# Autodesk Inventor assembly: Блок подъёма первога звена
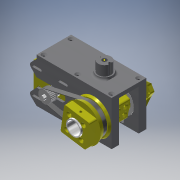
[picture p0: Inventor's stored thumbnail of the model, 180x180]
Saved by Autodesk Inventor 2019.1 (Build 231200000, 200)
## iProperties
Created: 2018-10-15
Part Number: Блок подъёма первога звена
Material: Типовые
Document SubType Name: Assembly
Designer: Олег
Author: Олег
## Documents named in this file (9)
- C:\Users\Олег\OneDrive\Общая\NoSpace 2.0\Манипулятор\Блок подъёма первога звена.iam
- C:\Users\Олег\OneDrive\Общая\NoSpace 2.0\Манипулятор\Основная часть подъемного механизма первого звена.iam
- C:\Users\Олег\OneDrive\Общая\NoSpace 2.0\Мотор-колесо\Мотор\Мотор.iam
- C:\Users\Олег\OneDrive\Общая\NoSpace 2.0\Манипулятор\Ось подъёмного блока первого звена.ipt
- C:\Users\Олег\OneDrive\Общая\NoSpace 2.0\Манипулятор\Переходник от первого звена к оси.ipt
- C:\Users\Олег\OneDrive\Общая\NoSpace 2.0\Манипулятор\Съёмное крепление мотора 37мм.ipt
- C:\Users\Олег\OneDrive\Общая\NoSpace 2.0\Манипулятор\Узел потенциометра.iam
- C:\Users\Олег\OneDrive\Общая\NoSpace 2.0\Манипулятор\Шкив.iam
- C:\Users\Олег\OneDrive\Общая\NoSpace 2.0\Манипулятор\Блок подъёма первога звена\Мастер проектирования\Передача с помощью зубчатых ремней4.iam
## Components (8 placed, 8 different names)
1. Основная часть подъемного механизма первого звена:1 [sub-assembly] — Совмещение:2, Совмещение:6, Заподлицо:1, Совмещение:8, Совмещение:9, Совмещение:10, Совмещение:11, Угол:1
2. Ось подъёмного блока первого звена:1 — Совмещение:6, Заподлицо:1, Совмещение:7, Совмещение:12, Заподлицо:2
3. Переходник от первого звена к оси:1 — Совмещение:7, Совмещение:8, Угол:2
4. Съёмное крепление мотора 37мм:1 — Совмещение:2, Совмещение:3, Совмещение:4, Совмещение:5, Угол:1
5. Узел потенциометра:1 [sub-assembly] — Совмещение:9, Совмещение:10, Совмещение:11
6. Шкив:1 [sub-assembly] — Совмещение:12, Заподлицо:2, Угол:2
7. Мотор:1 [sub-assembly] — Совмещение:3, Совмещение:4, Совмещение:5, Совмещение:13
8. Передача с помощью зубчатых ремней:1 [sub-assembly] — Совмещение:13
## Relationships (16: Mate 12, Flush 2, Angle 2)
- Совмещение:2 [Mate]: Основная часть подъемного механизма первого звена:1 ↔ Съёмное крепление мотора 37мм:1
- Совмещение:3 [Mate]: Съёмное крепление мотора 37мм:1 ↔ Мотор:1
- Совмещение:4 [Mate]: Съёмное крепление мотора 37мм:1 ↔ Мотор:1
- Совмещение:5 [Mate]: Съёмное крепление мотора 37мм:1 ↔ Мотор:1
- Совмещение:6 [Mate]: Основная часть подъемного механизма первого звена:1 ↔ Ось подъёмного блока первого звена:1
- Заподлицо:1 [Flush]: Основная часть подъемного механизма первого звена:1 ↔ Ось подъёмного блока первого звена:1
- Совмещение:7 [Mate]: Ось подъёмного блока первого звена:1 ↔ Переходник от первого звена к оси:1
- Совмещение:8 [Mate]: Основная часть подъемного механизма первого звена:1 ↔ Переходник от первого звена к оси:1
- Совмещение:9 [Mate]: Основная часть подъемного механизма первого звена:1 ↔ Узел потенциометра:1
- Совмещение:10 [Mate]: Основная часть подъемного механизма первого звена:1 ↔ Узел потенциометра:1
- Совмещение:11 [Mate]: Основная часть подъемного механизма первого звена:1 ↔ Узел потенциометра:1
- Совмещение:12 [Mate]: Ось подъёмного блока первого звена:1 ↔ Шкив:1
- Заподлицо:2 [Flush] (2 mm): Ось подъёмного блока первого звена:1 ↔ Шкив:1
- Совмещение:13 [Mate]: Мотор:1 ↔ Передача с помощью зубчатых ремней:1
- Угол:1 [Angle] (0 deg): Основная часть подъемного механизма первого звена:1 ↔ Съёмное крепление мотора 37мм:1
- Угол:2 [Angle] (0 deg): Переходник от первого звена к оси:1 ↔ Шкив:1
